# Autodesk Inventor assembly: EboxBottom
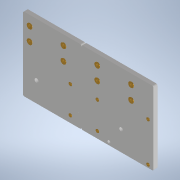
[picture p0: Inventor's stored thumbnail of the model, 180x180]
Saved by Autodesk Inventor 2021 (Build 250183000, 183)
## iProperties
Created: 2022-01-30
Part Number: EboxBottom
Document SubType Name: Assembly
Designer: Jorian Brusind
Author: Jorian Brusind
## Documents named in this file (5)
- C:\Users\Jorian Brusind\Documents\GitHub\HyperRail\Inventor Files\EboxBottom.iam
- C:\Users\Jorian Brusind\Documents\GitHub\HyperRail\Inventor Files\EboxBottom_1.ipt
- C:\Users\Jorian Brusind\Documents\GitHub\HyperRail\Inventor Files\EboxBottom_2.ipt
- C:\Users\Jorian Brusind\Documents\GitHub\HyperRail\Inventor Files\McMaster Files\Heat Inserts\M3-6mm-HeatInsert.ipt
- C:\Users\Jorian Brusind\Documents\GitHub\HyperRail\Inventor Files\McMaster Files\Heat Inserts\M5-6mm-HeatInsert.ipt
## Components (16 placed, 4 different names)
1. EboxBottom_1:1 — Flush:1, Flush:2, Mate:1, Mate:2, Mate:5, Mate:6, Mate:7, Mate:8, Mate:9, Flush:9, Flush:10, Flush:11, Flush:12, Flush:13, Flush:14
2. EboxBottom_2:1 — Flush:1, Flush:2, Mate:1, Mate:3, Mate:4, Mate:10, Mate:11, Mate:12, Mate:13, Mate:14, Mate:15, Flush:3, Flush:4, Flush:5, Flush:6, Flush:7, Flush:8, Flush:15, Flush:16
3. M3-6mm-HeatInsert:1 — Mate:2, Flush:13
4. M5-6mm-HeatInsert:1 — Mate:11, Flush:8
5. M5-6mm-HeatInsert:2 — Mate:6, Flush:9
6. M5-6mm-HeatInsert:3 — Mate:13, Flush:5
7. M5-6mm-HeatInsert:4 — Mate:12, Flush:7
8. M5-6mm-HeatInsert:5 — Mate:10, Flush:6
9. M5-6mm-HeatInsert:6 — Mate:9, Flush:11
10. M5-6mm-HeatInsert:7 — Mate:8, Flush:12
11. M5-6mm-HeatInsert:8 — Mate:7, Flush:10
12. M3-6mm-HeatInsert:2 — Mate:5, Flush:14
13. M3-6mm-HeatInsert:3 — Mate:3, Flush:15
14. M3-6mm-HeatInsert:4 — Mate:4, Flush:16
15. M3-6mm-HeatInsert:5 — Mate:15, Flush:3
16. M3-6mm-HeatInsert:6 — Mate:14, Flush:4
## Relationships (31: Flush 16, Mate 15)
- Flush:1: EboxBottom_1:1 ↔ EboxBottom_2:1
- Flush:2: EboxBottom_1:1 ↔ EboxBottom_2:1
- Mate:1: EboxBottom_1:1 ↔ EboxBottom_2:1
- Mate:2: EboxBottom_1:1 ↔ M3-6mm-HeatInsert:1
- Mate:3: EboxBottom_2:1 ↔ M3-6mm-HeatInsert:3
- Mate:4: EboxBottom_2:1 ↔ M3-6mm-HeatInsert:4
- Mate:5: EboxBottom_1:1 ↔ M3-6mm-HeatInsert:2
- Mate:6: EboxBottom_1:1 ↔ M5-6mm-HeatInsert:2
- Mate:7: EboxBottom_1:1 ↔ M5-6mm-HeatInsert:8
- Mate:8: EboxBottom_1:1 ↔ M5-6mm-HeatInsert:7
- Mate:9: EboxBottom_1:1 ↔ M5-6mm-HeatInsert:6
- Mate:10: EboxBottom_2:1 ↔ M5-6mm-HeatInsert:5
- Mate:11: EboxBottom_2:1 ↔ M5-6mm-HeatInsert:1
- Mate:12: EboxBottom_2:1 ↔ M5-6mm-HeatInsert:4
- Mate:13: EboxBottom_2:1 ↔ M5-6mm-HeatInsert:3
- Mate:14: EboxBottom_2:1 ↔ M3-6mm-HeatInsert:6
- Mate:15: EboxBottom_2:1 ↔ M3-6mm-HeatInsert:5
- Flush:3: EboxBottom_2:1 ↔ M3-6mm-HeatInsert:5
- Flush:4: EboxBottom_2:1 ↔ M3-6mm-HeatInsert:6
- Flush:5: EboxBottom_2:1 ↔ M5-6mm-HeatInsert:3
- Flush:6: EboxBottom_2:1 ↔ M5-6mm-HeatInsert:5
- Flush:7: EboxBottom_2:1 ↔ M5-6mm-HeatInsert:4
- Flush:8: EboxBottom_2:1 ↔ M5-6mm-HeatInsert:1
- Flush:9: EboxBottom_1:1 ↔ M5-6mm-HeatInsert:2
- Flush:10: EboxBottom_1:1 ↔ M5-6mm-HeatInsert:8
- Flush:11: EboxBottom_1:1 ↔ M5-6mm-HeatInsert:6
- Flush:12: EboxBottom_1:1 ↔ M5-6mm-HeatInsert:7
- Flush:13: EboxBottom_1:1 ↔ M3-6mm-HeatInsert:1
- Flush:14: EboxBottom_1:1 ↔ M3-6mm-HeatInsert:2
- Flush:15: EboxBottom_2:1 ↔ M3-6mm-HeatInsert:3
- Flush:16: EboxBottom_2:1 ↔ M3-6mm-HeatInsert:4
